# Autodesk Inventor assembly: PCBaseplateV2_PASLM_BSCoupled_NewPowell
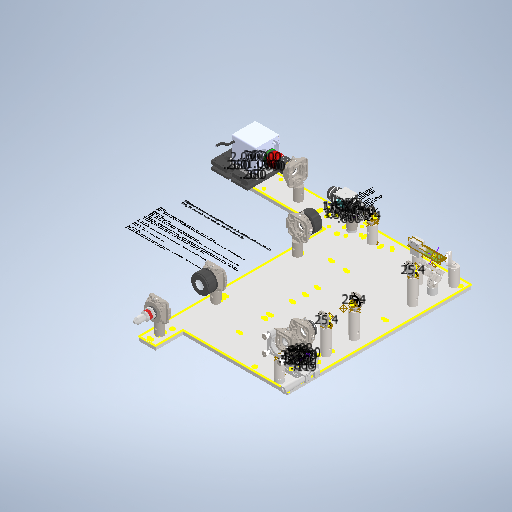
[picture p0: Inventor's stored thumbnail of the model, 512x512]
Saved by Autodesk Inventor 2025.2 (Build 292293000, 293)
## iProperties
Created: 2025-10-27
Part Number: PCBaseplateV2_PASLM_BSCoupled_NewPowell
Document SubType Name: Assembly
Designer: monolithic
Author: monolithic
## Documents named in this file (15)
- C:\Users\monolithic\Documents\GitHub\CAD\Monolith\John\Altair_PowellAndCylindricalBaseplatesCombined_10_16_2025\Assemblies\P_ASLM\PCBaseplateV2_PASLM_BSCoupled_NewPowell.iam
- C:\Users\monolithic\Documents\GitHub\CAD\Monolith\John\Altair_PowellBaseplate_SPIM_ASLM_CTASLM\Assembly\SubAssemblies\AC254-030-OnPost.iam
- C:\Users\monolithic\Documents\GitHub\CAD\Monolith\John\Altair_PowellBaseplate_SPIM_ASLM_CTASLM\Assembly\SubAssemblies\AC254-080-OnPost.iam
- C:\Users\monolithic\Documents\GitHub\CAD\Monolith\John\Altair_PowellBaseplate_SPIM_ASLM_CTASLM\Assembly\SubAssemblies\AC254-075-OnPost.iam
- C:\Users\monolithic\Documents\GitHub\CAD\Monolith\John\Altair_PowellBaseplate_SPIM_ASLM_CTASLM\Assembly\SubAssemblies\B1F-Mirror_OnPost.iam
- C:\Users\monolithic\Documents\GitHub\CAD\Monolith\John\Altair_PowellAndCylindricalBaseplatesCombined_10_16_2025\Assemblies\Subassemblies\Laser_OnPost.iam
- C:\Users\monolithic\Documents\GitHub\CAD\Monolith\John\Altair_PowellBaseplate_SPIM_ASLM_CTASLM\Assembly\SubAssemblies\AC254-300-OnPost.iam
- C:\Users\monolithic\Documents\GitHub\CAD\Monolith\John\Altair_PowellBaseplate_SPIM_ASLM_CTASLM\Assembly\SubAssemblies\ILO-Mounted.iam
- C:\Users\monolithic\Documents\GitHub\CAD\Monolith\John\Altair_PowellBaseplate_SPIM_ASLM_CTASLM\Assembly\SubAssemblies\TTL200-A-Mounted.iam
- C:\Users\monolithic\Documents\GitHub\CAD\Monolith\John\Altair_PowellBaseplate_SPIM_ASLM_CTASLM\Assembly\SubAssemblies\VoiceCoil_Assembly.iam
- C:\Users\monolithic\Documents\GitHub\CAD\Monolith\John\Altair_PowellBaseplate_SPIM_ASLM_CTASLM\Assembly\SubAssemblies\RFO-Mounted.iam
- C:\Users\monolithic\Documents\GitHub\CAD\Monolith\John\Altair_PowellAndCylindricalBaseplatesCombined_10_16_2025\Assemblies\Subassemblies\PowellLNR25M.iam
- C:\Users\monolithic\Documents\GitHub\CAD\Monolith\John\Altair_PowellAndCylindricalBaseplatesCombined_10_16_2025\Assemblies\Subassemblies\GalvoandK1s4.iam
- C:\Users\monolithic\Documents\GitHub\CAD\Monolith\John\Altair_PowellAndCylindricalBaseplatesCombined_10_16_2025\Assemblies\Subassemblies\BS_Assembly_Coupled_BSAdapterV9.iam
- C:\Users\monolithic\Documents\GitHub\CAD\Monolith\John\Altair_PowellAndCylindricalBaseplatesCombined_10_16_2025\Atlair_PowellandCylindrical_Baseplate_V5.ipt
## Components (16 placed, 14 different names)
1. Atlair_PowellandCylindrical_Baseplate_V5:2 — Mate:3, Mate:4, Mate:5, Mate:6, Angle:1, Mate:7, Mate:8, Mate:13, Mate:14, Angle:3, Mate:21, Mate:22, Mate:42, Angle:11, Mate:43, Mate:44, Mate:45
2. AC254-030-OnPost:1 [sub-assembly] — Mate:3, Mate:4
3. AC254-080-OnPost:1 [sub-assembly] — Mate:5, Mate:6, Angle:1
4. AC254-075-OnPost:1 [sub-assembly] — Mate:7, Mate:8
5. B1F-Mirror_OnPost:1 [sub-assembly] — Mate:13, Mate:14, Angle:3
6. Laser_OnPost:1 [sub-assembly] — Mate:21, Mate:22, Mate:25, Mate:26
7. Atlair_PowellandCylindrical_Baseplate_V5:1 — Mate:25, Mate:26, Mate:29, Mate:30, Angle:5, Mate:31, Mate:32, Angle:6, Mate:33, Mate:34, Mate:35, Mate:36, Angle:7, Mate:37, Angle:8, Mate:38, Mate:39, Mate:40, Angle:9, Mate:41, Angle:10, Mate:46
8. AC254-300-OnPost:1 [sub-assembly] — Mate:29, Mate:30, Angle:5
9. ILO-Mounted:1 [sub-assembly] — Mate:31, Mate:32, Angle:6
10. TTL200-A-Mounted:1 [sub-assembly] — Mate:33, Mate:34
11. TTL200-A-Mounted:2 [sub-assembly] — Mate:35, Mate:36, Angle:7
12. VoiceCoil_Assembly:1 [sub-assembly] — Mate:37, Angle:8, Mate:38
13. RFO-Mounted:1 [sub-assembly] — Mate:39, Mate:40, Angle:9
14. BS_Assembly_Coupled_BSAdapterV9:1 [sub-assembly] — Mate:41, Angle:10, Mate:42
15. PowellLNR25M:1 [sub-assembly] — Angle:11, Mate:43, Mate:44
16. GalvoandK1s4:1 [sub-assembly] — Mate:45, Mate:46
## Relationships (39: Mate 30, Angle 9)
- Mate:3: Atlair_PowellandCylindrical_Baseplate_V5:2 ↔ AC254-030-OnPost:1
- Mate:4: Atlair_PowellandCylindrical_Baseplate_V5:2 ↔ AC254-030-OnPost:1
- Mate:5: Atlair_PowellandCylindrical_Baseplate_V5:2 ↔ AC254-080-OnPost:1
- Mate:6: Atlair_PowellandCylindrical_Baseplate_V5:2 ↔ AC254-080-OnPost:1
- Angle:1 (90 deg): Atlair_PowellandCylindrical_Baseplate_V5:2 ↔ AC254-080-OnPost:1
- Mate:7: Atlair_PowellandCylindrical_Baseplate_V5:2 ↔ AC254-075-OnPost:1
- Mate:8: Atlair_PowellandCylindrical_Baseplate_V5:2 ↔ AC254-075-OnPost:1
- Mate:13: Atlair_PowellandCylindrical_Baseplate_V5:2 ↔ B1F-Mirror_OnPost:1
- Mate:14: Atlair_PowellandCylindrical_Baseplate_V5:2 ↔ B1F-Mirror_OnPost:1
- Angle:3 (45 deg): Atlair_PowellandCylindrical_Baseplate_V5:2 ↔ B1F-Mirror_OnPost:1
- Mate:21: Atlair_PowellandCylindrical_Baseplate_V5:2 ↔ Laser_OnPost:1
- Mate:22: Atlair_PowellandCylindrical_Baseplate_V5:2 ↔ Laser_OnPost:1
- Mate:25: Laser_OnPost:1 ↔ Atlair_PowellandCylindrical_Baseplate_V5:1
- Mate:26: Laser_OnPost:1 ↔ Atlair_PowellandCylindrical_Baseplate_V5:1
- Mate:29: Atlair_PowellandCylindrical_Baseplate_V5:1 ↔ AC254-300-OnPost:1
- Mate:30: Atlair_PowellandCylindrical_Baseplate_V5:1 ↔ AC254-300-OnPost:1
- Angle:5 (-90 deg): Atlair_PowellandCylindrical_Baseplate_V5:1 ↔ AC254-300-OnPost:1
- Mate:31: Atlair_PowellandCylindrical_Baseplate_V5:1 ↔ ILO-Mounted:1
- Mate:32: Atlair_PowellandCylindrical_Baseplate_V5:1 ↔ ILO-Mounted:1
- Angle:6 (180 deg): Atlair_PowellandCylindrical_Baseplate_V5:1 ↔ ILO-Mounted:1
- Mate:33: Atlair_PowellandCylindrical_Baseplate_V5:1 ↔ TTL200-A-Mounted:1
- Mate:34: Atlair_PowellandCylindrical_Baseplate_V5:1 ↔ TTL200-A-Mounted:1
- Mate:35: Atlair_PowellandCylindrical_Baseplate_V5:1 ↔ TTL200-A-Mounted:2
- Mate:36: Atlair_PowellandCylindrical_Baseplate_V5:1 ↔ TTL200-A-Mounted:2
- Angle:7 (180 deg): Atlair_PowellandCylindrical_Baseplate_V5:1 ↔ TTL200-A-Mounted:2
- Mate:37: Atlair_PowellandCylindrical_Baseplate_V5:1 ↔ VoiceCoil_Assembly:1
- Angle:8 (180 deg): Atlair_PowellandCylindrical_Baseplate_V5:1 ↔ VoiceCoil_Assembly:1
- Mate:38: Atlair_PowellandCylindrical_Baseplate_V5:1 ↔ VoiceCoil_Assembly:1
- Mate:39: Atlair_PowellandCylindrical_Baseplate_V5:1 ↔ RFO-Mounted:1
- Mate:40: Atlair_PowellandCylindrical_Baseplate_V5:1 ↔ RFO-Mounted:1
- Angle:9 (90 deg): Atlair_PowellandCylindrical_Baseplate_V5:1 ↔ RFO-Mounted:1
- Mate:41: Atlair_PowellandCylindrical_Baseplate_V5:1 ↔ BS_Assembly_Coupled_BSAdapterV9:1
- Angle:10 (90 deg): Atlair_PowellandCylindrical_Baseplate_V5:1 ↔ BS_Assembly_Coupled_BSAdapterV9:1
- Mate:42: Atlair_PowellandCylindrical_Baseplate_V5:2 ↔ BS_Assembly_Coupled_BSAdapterV9:1
- Angle:11 (-90 deg): Atlair_PowellandCylindrical_Baseplate_V5:2 ↔ PowellLNR25M:1
- Mate:43: Atlair_PowellandCylindrical_Baseplate_V5:2 ↔ PowellLNR25M:1
- Mate:44: Atlair_PowellandCylindrical_Baseplate_V5:2 ↔ PowellLNR25M:1
- Mate:45: Atlair_PowellandCylindrical_Baseplate_V5:2 ↔ GalvoandK1s4:1
- Mate:46: Atlair_PowellandCylindrical_Baseplate_V5:1 ↔ GalvoandK1s4:1
